# Autodesk Inventor assembly: newcutoutRotor
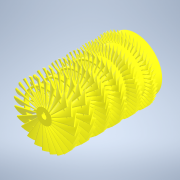
[picture p0: Inventor's stored thumbnail of the model, 180x180]
Saved by Autodesk Inventor 2021.2 (Build 252289000, 289)
## iProperties
Created: 2021-05-23
Part Number: newcutoutRotor
Document SubType Name: Assembly
Designer: Ryan
Author: Ryan
## Documents named in this file (7)
- C:\Users\Ryan\Documents\EDD\__NewCompressor\newcutoutRotor.iam
- C:\Users\Ryan\Documents\EDD\__NewCompressor\newRotor.24.1.0.ipt
- C:\Users\Ryan\Documents\EDD\__NewCompressor\newRotor.24.1.4.ipt
- C:\Users\Ryan\Documents\EDD\__NewCompressor\newRotor.36.1.8.ipt
- C:\Users\Ryan\Documents\EDD\__NewCompressor\newRotor.36.2.2.ipt
- C:\Users\Ryan\Documents\EDD\__NewCompressor\newRotor.48.2.6.ipt
- C:\Users\Ryan\Documents\EDD\__NewCompressor\newRotor.48.3.0.ipt
## Components (6 placed, 6 different names)
1. newRotor.24.1.0:1 — Insert:1
2. newRotor.24.1.4:1 — Insert:1, Insert:2
3. newRotor.36.1.8:1 — Insert:2, Insert:3
4. newRotor.36.2.2:1 — Insert:3, Insert:4
5. newRotor.48.2.6:1 — Insert:4, Insert:5
6. newRotor.48.3.0:1 — Insert:5
## Relationships (5: Insert 5)
- Insert:1: newRotor.24.1.0:1 ↔ newRotor.24.1.4:1
- Insert:2: newRotor.24.1.4:1 ↔ newRotor.36.1.8:1
- Insert:3: newRotor.36.1.8:1 ↔ newRotor.36.2.2:1
- Insert:4: newRotor.36.2.2:1 ↔ newRotor.48.2.6:1
- Insert:5: newRotor.48.2.6:1 ↔ newRotor.48.3.0:1
